# Autodesk Inventor assembly: Trasmissione cinghie - Taglio
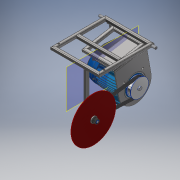
[picture p0: Inventor's stored thumbnail of the model, 180x180]
Saved by Autodesk Inventor 2018 (Build 220112000, 112)
## iProperties
Created: 2020-06-04
Part Number: Trasmissione cinghie - Taglio
Material: Generico
Document SubType Name: Assembly
Designer: Francesco
Mass: 11579.7 g
Surface Area: 9613.4 cm^2
Volume: 5451 cm^3
Density: 2.12433 g/cm^3
Author: Francesco
## Documents named in this file (13)
- C:\Users\Francesco\no-brim\Meccanica\Progetto Inventor no-brim\Assiemi\Trasmissione cinghie - Taglio.iam
- C:\Users\Francesco\no-brim\Meccanica\Progetto Inventor no-brim\Parti\Puleggia maggiore.ipt
- C:\Users\Francesco\no-brim\Meccanica\Progetto Inventor no-brim\Parti\Puleggia minore.ipt
- C:\Users\Francesco\no-brim\Meccanica\Progetto Inventor no-brim\Parti\Cinghia.ipt
- C:\Users\Francesco\no-brim\Meccanica\Progetto Inventor no-brim\Parti\Sega Circolare 300 mm.ipt
- C:\Users\Francesco\no-brim\Meccanica\Progetto Inventor no-brim\Parti\Motorredutor Bonfiglioli .iam
- C:\Users\Francesco\no-brim\Meccanica\Progetto Inventor no-brim\Parti\Lamiera supporto motore.ipt
- C:\Users\Francesco\no-brim\Meccanica\Progetto Inventor no-brim\Assiemi\Telaietto trasmissione - Taglio.iam
- C:\Users\Francesco\no-brim\Meccanica\Progetto Inventor no-brim\Parti\Distanziale lama.ipt
- C:\Users\Francesco\no-brim\Meccanica\Progetto Inventor no-brim\Unificati\it-IT\UNI 8836\UNI 8836 - 21,4 x 38 - 4,6.ipt
- C:\Users\Francesco\no-brim\Meccanica\Progetto Inventor no-brim\Unificati\it-IT\ISO 7043\ISO 7043 - M16 - ISO.ipt
- C:\Users\Francesco\no-brim\Meccanica\Progetto Inventor no-brim\Unificati\it-IT\SKF B - angular contact\SKF B7204 BE.ipt
- C:\Users\Francesco\no-brim\Meccanica\Progetto Inventor no-brim\Parti\Porta cuscinetto puleggia operatrice.ipt
## Components (12 placed, 12 different names)
1. Puleggia maggiore:1 — Allineato:1, Coincidente:2, Coincidente:3, Coincidente:11, Angolo:1, Coincidente:15
2. Puleggia minore:1 — Allineato:1, Coincidente:1, Coincidente:4, Coincidente:17, Coincidente:18, Coincidente:19, Coincidente:21, Coincidente:23, Coincidente:27, Coincidente:28
3. Cinghia:1 — Coincidente:1, Coincidente:2, Coincidente:3
4. Sega Circolare 300 mm:1 — Coincidente:4, Coincidente:20, Coincidente:22
5. Lamiera supporto motore:1 — Coincidente:11, Angolo:1, Coincidente:13, Coincidente:14, Angolo:2, Coincidente:16, Allineato:6, Allineato:7
6. Motorredutor Bonfiglioli :1 [sub-assembly] — Coincidente:13, Coincidente:14, Angolo:2, Coincidente:15
7. Telaietto trasmissione:1 [sub-assembly] — Allineato:5, Coincidente:16, Allineato:6, Allineato:7, Coincidente:17, Coincidente:29
8. Distanziale lama:1 — Coincidente:18, Coincidente:19, Coincidente:20
9. UNI 8836 21,4 x 38:1 — Coincidente:21, Coincidente:22, Coincidente:24
10. ISO 7043 M16:1 — Coincidente:23, Coincidente:24
11. SKF B- Contatto angolare SKF B7204 BE:1 — Coincidente:25, Coincidente:26, Coincidente:27
12. Porta cuscinetto puleggia operatrice:1 — Coincidente:25, Coincidente:26, Coincidente:28, Coincidente:29
## Relationships (28: Mate 22, Flush 4, Angle 2)
- Allineato:1 [Flush]: Puleggia maggiore:1 ↔ Puleggia minore:1
- Coincidente:1 [Mate]: Puleggia minore:1 ↔ Cinghia:1
- Coincidente:2 [Mate]: Puleggia maggiore:1 ↔ Cinghia:1
- Coincidente:3 [Mate] (1.5 mm): Puleggia maggiore:1 ↔ Cinghia:1
- Coincidente:4 [Mate]: Puleggia minore:1 ↔ Sega Circolare 300 mm:1
- Coincidente:11 [Mate]: Puleggia maggiore:1 ↔ Lamiera supporto motore:1
- Angolo:1 [Angle] (0 deg): Puleggia maggiore:1 ↔ Lamiera supporto motore:1
- Coincidente:13 [Mate]: Lamiera supporto motore:1 ↔ Motorredutor Bonfiglioli :1
- Coincidente:14 [Mate]: Lamiera supporto motore:1 ↔ Motorredutor Bonfiglioli :1
- Angolo:2 [Angle] (-90 deg): Lamiera supporto motore:1 ↔ Motorredutor Bonfiglioli :1
- Coincidente:15 [Mate]: Puleggia maggiore:1 ↔ Motorredutor Bonfiglioli :1
- Allineato:5 [Flush] (-150 mm): Telaietto trasmissione:1
- Coincidente:16 [Mate]: Lamiera supporto motore:1 ↔ Telaietto trasmissione:1
- Allineato:6 [Flush]: Lamiera supporto motore:1 ↔ Telaietto trasmissione:1
- Allineato:7 [Flush]: Lamiera supporto motore:1 ↔ Telaietto trasmissione:1
- Coincidente:17 [Mate] (210 mm): Puleggia minore:1 ↔ Telaietto trasmissione:1
- Coincidente:18 [Mate]: Puleggia minore:1 ↔ Distanziale lama:1
- Coincidente:19 [Mate]: Puleggia minore:1 ↔ Distanziale lama:1
- Coincidente:20 [Mate]: Sega Circolare 300 mm:1 ↔ Distanziale lama:1
- Coincidente:21 [Mate]: Puleggia minore:1 ↔ UNI 8836 21,4 x 38:1
- Coincidente:22 [Mate]: Sega Circolare 300 mm:1 ↔ UNI 8836 21,4 x 38:1
- Coincidente:23 [Mate]: Puleggia minore:1 ↔ ISO 7043 M16:1
- Coincidente:24 [Mate]: UNI 8836 21,4 x 38:1 ↔ ISO 7043 M16:1
- Coincidente:25 [Mate]: SKF B- Contatto angolare SKF B7204 BE:1 ↔ Porta cuscinetto puleggia operatrice:1
- Coincidente:26 [Mate]: SKF B- Contatto angolare SKF B7204 BE:1 ↔ Porta cuscinetto puleggia operatrice:1
- Coincidente:27 [Mate]: Puleggia minore:1 ↔ SKF B- Contatto angolare SKF B7204 BE:1
- Coincidente:28 [Mate] (5 mm): Puleggia minore:1 ↔ Porta cuscinetto puleggia operatrice:1
- Coincidente:29 [Mate]: Telaietto trasmissione:1 ↔ Porta cuscinetto puleggia operatrice:1
